# Autodesk Inventor assembly: sestaveny dum
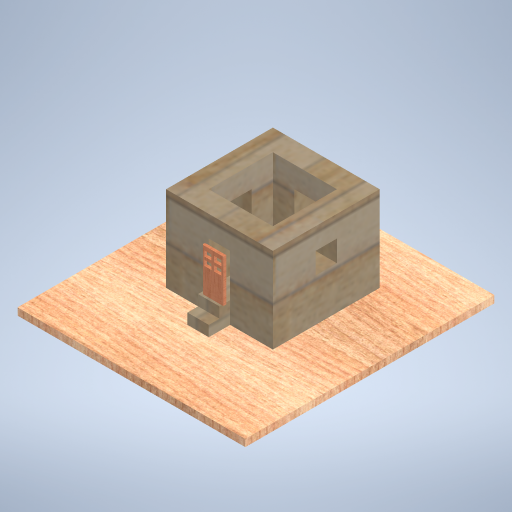
[picture p0: Inventor's stored thumbnail of the model, 512x512]
Saved by Autodesk Inventor 2023 (Build 270158000, 158)
## iProperties
Created: 2022-10-19
Part Number: sestaveny dum
Document SubType Name: Assembly
Designer: zak
Author: zak
## Documents named in this file (4)
- H:\KYB\minecraft baracek\model domu\sestaveny dum.iam
- H:\KYB\minecraft baracek\model domu\deska.ipt
- H:\KYB\minecraft baracek\model domu\steny.ipt
- H:\KYB\minecraft baracek\model domu\dvere.ipt
## Components (3 placed, 3 different names)
1. deska:1 — Proti sobě:1
2. steny:1 — Proti sobě:1, Proti sobě:2
3. dvere:1 — Proti sobě:2
## Relationships (2: Mate 2)
- Proti sobě:1 [Mate]: deska:1 ↔ steny:1
- Proti sobě:2 [Mate]: steny:1 ↔ dvere:1
